# Autodesk Inventor assembly: LR_02
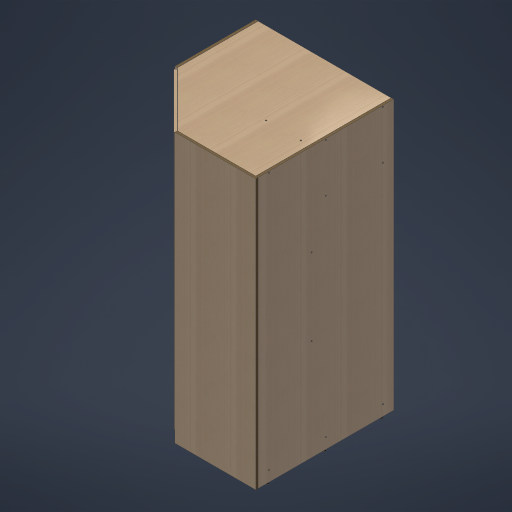
[picture p0: Inventor's stored thumbnail of the model, 512x512]
Saved by Autodesk Inventor 2024.3 (Build 283343000, 343)
## iProperties
Created: 2013-04-02
Part Number: LR_02
Document SubType Name: Assembly
Designer: User
Description: Corner Cabinet
Author: User
## Documents named in this file (23)
- C:\W4INV 2024 Design\PROJECTS\Living Room\Corner Cabinet\LR_02.iam
- C:\W4INV 2024 Design\PROJECTS\Samples\Living Room\Corner Cabinet\LR_0200.ipt
- C:\W4INV 2024 Design\PROJECTS\Samples\Living Room\Corner Cabinet\LR_0203.ipt
- C:\W4INV 2024 Design\PROJECTS\Samples\Living Room\Corner Cabinet\LR_0206.ipt
- C:\W4INV 2024 Design\PROJECTS\Samples\Living Room\Corner Cabinet\LR_0210.ipt
- C:\W4INV 2024 Design\PROJECTS\Samples\Living Room\Corner Cabinet\LR_0201.ipt
- C:\W4INV 2024 Design\PROJECTS\Samples\Living Room\Corner Cabinet\LR_0209.ipt
- C:\W4INV 2024 Design\PROJECTS\Samples\Living Room\Corner Cabinet\LR_0204.ipt
- C:\W4INV 2024 Design\PROJECTS\Samples\Living Room\Corner Cabinet\LR_0205.ipt
- C:\W4INV 2024 Design\PROJECTS\Samples\Living Room\Corner Cabinet\LR_0208.ipt
- C:\W4INV 2024 Design\PROJECTS\Samples\Living Room\Corner Cabinet\LR_0202.ipt
- C:\W4INV 2024 Design\PROJECTS\Samples\Living Room\Corner Cabinet\LR_0207.ipt
- C:\W4INV 2024 Design\_LIBRARY\Fixed joints\Confirmat\CONFIRMAT\Confirmat L50 & Cap D10 NB T18 PB T 18.ipt
- C:\W4INV 2024 Design\_LIBRARY\Fixed joints\Minifix joint\MINIFIX D15 v2\Minifix D15 & Dowel L34 & Cap D15 PB T18 LH.ipt
- C:\W4INV 2024 Design\_LIBRARY\Fixed joints\Minifix joint\MINIFIX D15 v2\Minifix D15 & Dowel L34 & Cap D15 PB T18 RH.ipt
- C:\W4INV 2024 Design\_LIBRARY\Hinges\45 DEGREE HINGE\45 Degree Hinge with Wood Screws And Cup Fixing Wood Screws.iam
- C:\W4INV 2024 Design\_LIBRARY\Supports and legs\Supports\ADJUSTABLE SUPPORT\Support M6 H27 D18 with Bushing SB T18.ipt
- C:\W4INV 2023 Design\LIBRARY\Fixed joints\Confirmat\CONFIRMAT.ipt
- C:\W4INV 2023 Design\LIBRARY\Holders\Shelf holder D5.ipt
- C:\W4INV 2023 Design\LIBRARY\Supports and legs\Supports\ADJUSTABLE SUPPORT.ipt
- C:\W4INV 2023 Design\LIBRARY\Fixed joints\Minifix joint\MINIFIX D15 v2.ipt
- C:\W4INV 2023 Design\LIBRARY\Hinges\45 DEGREE HINGE.iam
- C:\W4INV 2024 Design\_LIBRARY\Holders\Shelf holder D5\Shelf support D5 L16 HOL 3 CAP ON.ipt
## Components (68 placed, 17 different names)
1. LR_0200-Right Side:1 — Flush:1, Flush:2, Mate:135, Mate:141, Mate:180, Mate:188, Mate:192, Mate:200
2. LR_0203-Left Side:1 — Flush:3, Flush:4, Mate:144, Flush:64, Mate:146, Flush:65, Mate:154, Mate:158, Mate:162, Mate:166, Mate:170, Mate:174, Flush:96, Mate:208, Flush:97, Mate:210, Flush:98, Mate:212, Flush:99, Mate:214
3. LR_0206-Back:1 — Mate:91, Flush:38, Mate:93, Flush:39, Mate:95, Flush:40, Mate:97, Flush:41, Mate:99, Flush:42, Mate:101, Flush:43, Flush:48, Flush:49, Mate:115, Flush:50, Mate:117, Flush:51, Mate:147, Mate:148, Flush:66, Mate:149, Mate:150, Flush:67, Mate:151, Mate:152, Flush:68
4. LR_0210-Top:1 — Mate:92, Mate:96, Mate:100, Flush:46, Flush:47, Flush:69, Flush:75, Flush:82, Flush:88
5. LR_0201-Bottom:1 — Mate:94, Mate:98, Mate:102, Flush:73, Flush:79, Flush:86, Flush:92, Flush:93, Flush:95
6. LR_0209-Vertical Partiton:1 — Flush:5, Mate:108, Mate:110, Mate:112, Mate:114, Mate:132, Mate:138, Mate:202, Mate:205
7. LR_0204-Shelve:1 — Mate:116, Mate:118, Flush:71, Flush:77
8. LR_0208-Left Back:1
9. LR_0202-Door:1 — Mate:71, Angle:2, Mate:72, Mate:73, Mate:74
10. LR_0207-Plynth:1
11. Confirmat L50 & Cap D10 NB T18 PB T 18:1 — Mate:91, Mate:92, Flush:38
12. Confirmat L50 & Cap D10 NB T18 PB T 18:2 — Mate:93, Mate:94, Flush:39
13. Confirmat L50 & Cap D10 NB T18 PB T 18:3 — Mate:95, Mate:96, Flush:40
14. Confirmat L50 & Cap D10 NB T18 PB T 18:4 — Mate:97, Mate:98, Flush:41
15. Confirmat L50 & Cap D10 NB T18 PB T 18:5 — Mate:99, Mate:100, Flush:42
16. Confirmat L50 & Cap D10 NB T18 PB T 18:6 — Mate:101, Mate:102, Flush:43
17. Confirmat L50 & Cap D10 NB T18 PB T 18:9 — Mate:107, Flush:46, Mate:108
18. Confirmat L50 & Cap D10 NB T18 PB T 18:10 — Mate:109, Flush:47, Mate:110
19. Confirmat L50 & Cap D10 NB T18 PB T 18:11 — Mate:111, Flush:48, Mate:112
20. Confirmat L50 & Cap D10 NB T18 PB T 18:12 — Mate:113, Flush:49, Mate:114
21. Confirmat L50 & Cap D10 NB T18 PB T 18:13 — Mate:115, Flush:50, Mate:116
22. Confirmat L50 & Cap D10 NB T18 PB T 18:14 — Mate:117, Flush:51, Mate:118
23. Support M6 H27 D18 with Bushing SB T18:6 — Mate:143, Mate:144, Flush:64
24. Support M6 H27 D18 with Bushing SB T18:7 — Mate:145, Mate:146, Flush:65
25. Support M6 H27 D18 with Bushing SB T18:8 — Mate:147, Mate:148, Flush:66
26. Support M6 H27 D18 with Bushing SB T18:9 — Mate:149, Mate:150, Flush:67
27. Support M6 H27 D18 with Bushing SB T18:10 — Mate:151, Mate:152, Flush:68
28. Minifix D15 & Dowel L34 & Cap D15 PB T18 LH:1 — Mate:153, Flush:69, Mate:154
29. Minifix D15 & Dowel L34 & Cap D15 PB T18 RH:3 — Mate:157, Flush:71, Mate:158
30. Minifix D15 & Dowel L34 & Cap D15 PB T18 RH:5 — Mate:161, Flush:73, Mate:162
31. Minifix D15 & Dowel L34 & Cap D15 PB T18 LH:7 — Mate:165, Flush:75, Mate:166
32. Minifix D15 & Dowel L34 & Cap D15 PB T18 LH:9 — Mate:169, Flush:77, Mate:170
33. Minifix D15 & Dowel L34 & Cap D15 PB T18 LH:11 — Mate:173, Flush:79, Mate:174
34. Minifix D15 & Dowel L34 & Cap D15 PB T18 LH:14 — Mate:179, Flush:82, Mate:180
35. Minifix D15 & Dowel L34 & Cap D15 PB T18 RH:18 — Mate:187, Flush:86, Mate:188
36. Minifix D15 & Dowel L34 & Cap D15 PB T18 RH:20 — Mate:191, Flush:88, Mate:192
37. Minifix D15 & Dowel L34 & Cap D15 PB T18 LH:24 — Mate:199, Flush:92, Mate:200
38. Confirmat L50 & Cap D10 NB T18 PB T 18:15 — Mate:201, Flush:93, Mate:202
39. Confirmat L50 & Cap D10 NB T18 PB T 18:17 — Flush:95, Mate:205, Mate:206
40. 45 Degree Hinge with Wood Screws And Cup Fixing Wood Screws:2 [sub-assembly] — Mate:207, Flush:96, Mate:208
41. 45 Degree Hinge with Wood Screws And Cup Fixing Wood Screws:3 [sub-assembly] — Mate:209, Flush:97, Mate:210
42. 45 Degree Hinge with Wood Screws And Cup Fixing Wood Screws:4 [sub-assembly] — Mate:211, Flush:98, Mate:212
43. 45 Degree Hinge with Wood Screws And Cup Fixing Wood Screws:5 [sub-assembly] — Mate:213, Flush:99, Mate:214
44. LR_0205-Shelve:1 — Mate:133, Mate:136, Mate:139, Mate:142
45. Shelf support D5 L16 HOL 3 CAP ON:1 — Mate:131, Mate:132, Mate:133
46. Shelf support D5 L16 HOL 3 CAP ON:3 — Mate:137, Mate:138, Mate:139
47. Shelf support D5 L16 HOL 3 CAP ON:4 — Mate:140, Mate:141, Mate:142
48. Shelf support D5 L16 HOL 3 CAP ON:2 — Mate:134, Mate:135, Mate:136
49. LR_0205-Shelve:2
50. Shelf support D5 L16 HOL 3 CAP ON:5
51. Shelf support D5 L16 HOL 3 CAP ON:6
52. Shelf support D5 L16 HOL 3 CAP ON:7
53. Shelf support D5 L16 HOL 3 CAP ON:8
54. LR_0205-Shelve:3
55. Shelf support D5 L16 HOL 3 CAP ON:9
56. Shelf support D5 L16 HOL 3 CAP ON:10
57. Shelf support D5 L16 HOL 3 CAP ON:11
58. Shelf support D5 L16 HOL 3 CAP ON:12
59. LR_0205-Shelve:4
60. Shelf support D5 L16 HOL 3 CAP ON:13
61. Shelf support D5 L16 HOL 3 CAP ON:14
62. Shelf support D5 L16 HOL 3 CAP ON:15
63. Shelf support D5 L16 HOL 3 CAP ON:16
64. LR_0205-Shelve:5
65. Shelf support D5 L16 HOL 3 CAP ON:17
66. Shelf support D5 L16 HOL 3 CAP ON:18
67. Shelf support D5 L16 HOL 3 CAP ON:19
68. Shelf support D5 L16 HOL 3 CAP ON:20
## Component patterns: (5 elements, first: LR_0205-Shelve:1 + Shelf support D5 L16 HOL 3 CAP ON:1 + Shelf support D5 L16 HOL 3 CAP ON:3 + Shelf support D5 L16 HOL 3 CAP ON:4 + Shelf support D5 L16 HOL 3 CAP ON:2)
## Relationships (124: Mate 82, Flush 38, Angle 4)
- Flush:1 (-80 mm): LR_0200-Right Side:1
- Flush:2 (-80 mm): LR_0200-Right Side:1
- Flush:3 (-80 mm): LR_0203-Left Side:1
- Flush:4 (-80 mm): LR_0203-Left Side:1
- Flush:5 (-80 mm): LR_0209-Vertical Partiton:1
- Mate:71: LR_0202-Door:1
- Angle:2 (0 deg): LR_0202-Door:1
- Mate:72: LR_0202-Door:1
- Angle:3 (0 deg)
- Mate:73: LR_0202-Door:1
- Angle:4 (0 deg)
- Mate:74: LR_0202-Door:1
- Angle:5 (0 deg)
- Mate:91: LR_0206-Back:1 ↔ Confirmat L50 & Cap D10 NB T18 PB T 18:1
- Mate:92 (-9 mm): LR_0210-Top:1 ↔ Confirmat L50 & Cap D10 NB T18 PB T 18:1
- Flush:38: LR_0206-Back:1 ↔ Confirmat L50 & Cap D10 NB T18 PB T 18:1
- Mate:93: LR_0206-Back:1 ↔ Confirmat L50 & Cap D10 NB T18 PB T 18:2
- Mate:94 (-9 mm): LR_0201-Bottom:1 ↔ Confirmat L50 & Cap D10 NB T18 PB T 18:2
- Flush:39: LR_0206-Back:1 ↔ Confirmat L50 & Cap D10 NB T18 PB T 18:2
- Mate:95: LR_0206-Back:1 ↔ Confirmat L50 & Cap D10 NB T18 PB T 18:3
- Mate:96 (-9 mm): LR_0210-Top:1 ↔ Confirmat L50 & Cap D10 NB T18 PB T 18:3
- Flush:40: LR_0206-Back:1 ↔ Confirmat L50 & Cap D10 NB T18 PB T 18:3
- Mate:97: LR_0206-Back:1 ↔ Confirmat L50 & Cap D10 NB T18 PB T 18:4
- Mate:98 (-9 mm): LR_0201-Bottom:1 ↔ Confirmat L50 & Cap D10 NB T18 PB T 18:4
- Flush:41: LR_0206-Back:1 ↔ Confirmat L50 & Cap D10 NB T18 PB T 18:4
- Mate:99: LR_0206-Back:1 ↔ Confirmat L50 & Cap D10 NB T18 PB T 18:5
- Mate:100 (-9 mm): LR_0210-Top:1 ↔ Confirmat L50 & Cap D10 NB T18 PB T 18:5
- Flush:42: LR_0206-Back:1 ↔ Confirmat L50 & Cap D10 NB T18 PB T 18:5
- Mate:101: LR_0206-Back:1 ↔ Confirmat L50 & Cap D10 NB T18 PB T 18:6
- Mate:102 (-9 mm): LR_0201-Bottom:1 ↔ Confirmat L50 & Cap D10 NB T18 PB T 18:6
- Flush:43: LR_0206-Back:1 ↔ Confirmat L50 & Cap D10 NB T18 PB T 18:6
- Mate:107: Confirmat L50 & Cap D10 NB T18 PB T 18:9
- Flush:46: LR_0210-Top:1 ↔ Confirmat L50 & Cap D10 NB T18 PB T 18:9
- Mate:108 (-9 mm): LR_0209-Vertical Partiton:1 ↔ Confirmat L50 & Cap D10 NB T18 PB T 18:9
- Mate:109: Confirmat L50 & Cap D10 NB T18 PB T 18:10
- Flush:47: LR_0210-Top:1 ↔ Confirmat L50 & Cap D10 NB T18 PB T 18:10
- Mate:110 (-9 mm): LR_0209-Vertical Partiton:1 ↔ Confirmat L50 & Cap D10 NB T18 PB T 18:10
- Mate:111: Confirmat L50 & Cap D10 NB T18 PB T 18:11
- Flush:48: LR_0206-Back:1 ↔ Confirmat L50 & Cap D10 NB T18 PB T 18:11
- Mate:112 (-9 mm): LR_0209-Vertical Partiton:1 ↔ Confirmat L50 & Cap D10 NB T18 PB T 18:11
- Mate:113: Confirmat L50 & Cap D10 NB T18 PB T 18:12
- Flush:49: LR_0206-Back:1 ↔ Confirmat L50 & Cap D10 NB T18 PB T 18:12
- Mate:114 (-9 mm): LR_0209-Vertical Partiton:1 ↔ Confirmat L50 & Cap D10 NB T18 PB T 18:12
- Mate:115: LR_0206-Back:1 ↔ Confirmat L50 & Cap D10 NB T18 PB T 18:13
- Flush:50: LR_0206-Back:1 ↔ Confirmat L50 & Cap D10 NB T18 PB T 18:13
- Mate:116 (-9 mm): LR_0204-Shelve:1 ↔ Confirmat L50 & Cap D10 NB T18 PB T 18:13
- Mate:117: LR_0206-Back:1 ↔ Confirmat L50 & Cap D10 NB T18 PB T 18:14
- Flush:51: LR_0206-Back:1 ↔ Confirmat L50 & Cap D10 NB T18 PB T 18:14
- Mate:118 (-9 mm): LR_0204-Shelve:1 ↔ Confirmat L50 & Cap D10 NB T18 PB T 18:14
- Mate:131: Shelf support D5 L16 HOL 3 CAP ON:1
- Mate:132: LR_0209-Vertical Partiton:1 ↔ Shelf support D5 L16 HOL 3 CAP ON:1
- Mate:133 (2.5 mm): LR_0205-Shelve:1 ↔ Shelf support D5 L16 HOL 3 CAP ON:1
- Mate:134: Shelf support D5 L16 HOL 3 CAP ON:2
- Mate:135: LR_0200-Right Side:1 ↔ Shelf support D5 L16 HOL 3 CAP ON:2
- Mate:136 (2.5 mm): LR_0205-Shelve:1 ↔ Shelf support D5 L16 HOL 3 CAP ON:2
- Mate:137: Shelf support D5 L16 HOL 3 CAP ON:3
- Mate:138: LR_0209-Vertical Partiton:1 ↔ Shelf support D5 L16 HOL 3 CAP ON:3
- Mate:139 (2.5 mm): LR_0205-Shelve:1 ↔ Shelf support D5 L16 HOL 3 CAP ON:3
- Mate:140: Shelf support D5 L16 HOL 3 CAP ON:4
- Mate:141: LR_0200-Right Side:1 ↔ Shelf support D5 L16 HOL 3 CAP ON:4
- Mate:142 (2.5 mm): LR_0205-Shelve:1 ↔ Shelf support D5 L16 HOL 3 CAP ON:4
- Mate:143: Support M6 H27 D18 with Bushing SB T18:6
- Mate:144 (17.5 mm): LR_0203-Left Side:1 ↔ Support M6 H27 D18 with Bushing SB T18:6
- Flush:64 (9 mm): LR_0203-Left Side:1 ↔ Support M6 H27 D18 with Bushing SB T18:6
- Mate:145: Support M6 H27 D18 with Bushing SB T18:7
- Mate:146 (17.5 mm): LR_0203-Left Side:1 ↔ Support M6 H27 D18 with Bushing SB T18:7
- Flush:65 (9 mm): LR_0203-Left Side:1 ↔ Support M6 H27 D18 with Bushing SB T18:7
- Mate:147: LR_0206-Back:1 ↔ Support M6 H27 D18 with Bushing SB T18:8
- Mate:148 (17.5 mm): LR_0206-Back:1 ↔ Support M6 H27 D18 with Bushing SB T18:8
- Flush:66 (9 mm): LR_0206-Back:1 ↔ Support M6 H27 D18 with Bushing SB T18:8
- Mate:149: LR_0206-Back:1 ↔ Support M6 H27 D18 with Bushing SB T18:9
- Mate:150 (17.5 mm): LR_0206-Back:1 ↔ Support M6 H27 D18 with Bushing SB T18:9
- Flush:67 (9 mm): LR_0206-Back:1 ↔ Support M6 H27 D18 with Bushing SB T18:9
- Mate:151: LR_0206-Back:1 ↔ Support M6 H27 D18 with Bushing SB T18:10
- Mate:152 (17.5 mm): LR_0206-Back:1 ↔ Support M6 H27 D18 with Bushing SB T18:10
- Flush:68 (9 mm): LR_0206-Back:1 ↔ Support M6 H27 D18 with Bushing SB T18:10
- Mate:153: Minifix D15 & Dowel L34 & Cap D15 PB T18 LH:1
- Flush:69 (18 mm): LR_0210-Top:1 ↔ Minifix D15 & Dowel L34 & Cap D15 PB T18 LH:1
- Mate:154: LR_0203-Left Side:1 ↔ Minifix D15 & Dowel L34 & Cap D15 PB T18 LH:1
- Mate:157: Minifix D15 & Dowel L34 & Cap D15 PB T18 RH:3
- Flush:71 (18 mm): LR_0204-Shelve:1 ↔ Minifix D15 & Dowel L34 & Cap D15 PB T18 RH:3
- Mate:158: LR_0203-Left Side:1 ↔ Minifix D15 & Dowel L34 & Cap D15 PB T18 RH:3
- Mate:161: Minifix D15 & Dowel L34 & Cap D15 PB T18 RH:5
- Flush:73 (18 mm): LR_0201-Bottom:1 ↔ Minifix D15 & Dowel L34 & Cap D15 PB T18 RH:5
- Mate:162: LR_0203-Left Side:1 ↔ Minifix D15 & Dowel L34 & Cap D15 PB T18 RH:5
- Mate:165: Minifix D15 & Dowel L34 & Cap D15 PB T18 LH:7
- Flush:75 (18 mm): LR_0210-Top:1 ↔ Minifix D15 & Dowel L34 & Cap D15 PB T18 LH:7
- Mate:166: LR_0203-Left Side:1 ↔ Minifix D15 & Dowel L34 & Cap D15 PB T18 LH:7
- Mate:169: Minifix D15 & Dowel L34 & Cap D15 PB T18 LH:9
- Flush:77 (18 mm): LR_0204-Shelve:1 ↔ Minifix D15 & Dowel L34 & Cap D15 PB T18 LH:9
- Mate:170: LR_0203-Left Side:1 ↔ Minifix D15 & Dowel L34 & Cap D15 PB T18 LH:9
- Mate:173: Minifix D15 & Dowel L34 & Cap D15 PB T18 LH:11
- Flush:79 (18 mm): LR_0201-Bottom:1 ↔ Minifix D15 & Dowel L34 & Cap D15 PB T18 LH:11
- Mate:174: LR_0203-Left Side:1 ↔ Minifix D15 & Dowel L34 & Cap D15 PB T18 LH:11
- Mate:179: Minifix D15 & Dowel L34 & Cap D15 PB T18 LH:14
- Flush:82 (18 mm): LR_0210-Top:1 ↔ Minifix D15 & Dowel L34 & Cap D15 PB T18 LH:14
- Mate:180: LR_0200-Right Side:1 ↔ Minifix D15 & Dowel L34 & Cap D15 PB T18 LH:14
- Mate:187: Minifix D15 & Dowel L34 & Cap D15 PB T18 RH:18
- Flush:86 (18 mm): LR_0201-Bottom:1 ↔ Minifix D15 & Dowel L34 & Cap D15 PB T18 RH:18
- Mate:188: LR_0200-Right Side:1 ↔ Minifix D15 & Dowel L34 & Cap D15 PB T18 RH:18
- Mate:191: Minifix D15 & Dowel L34 & Cap D15 PB T18 RH:20
- Flush:88 (18 mm): LR_0210-Top:1 ↔ Minifix D15 & Dowel L34 & Cap D15 PB T18 RH:20
- Mate:192: LR_0200-Right Side:1 ↔ Minifix D15 & Dowel L34 & Cap D15 PB T18 RH:20
- Mate:199: Minifix D15 & Dowel L34 & Cap D15 PB T18 LH:24
- Flush:92 (18 mm): LR_0201-Bottom:1 ↔ Minifix D15 & Dowel L34 & Cap D15 PB T18 LH:24
- Mate:200: LR_0200-Right Side:1 ↔ Minifix D15 & Dowel L34 & Cap D15 PB T18 LH:24
- Mate:201: Confirmat L50 & Cap D10 NB T18 PB T 18:15
- Flush:93: LR_0201-Bottom:1 ↔ Confirmat L50 & Cap D10 NB T18 PB T 18:15
- Mate:202 (-9 mm): LR_0209-Vertical Partiton:1 ↔ Confirmat L50 & Cap D10 NB T18 PB T 18:15
- Flush:95: LR_0201-Bottom:1 ↔ Confirmat L50 & Cap D10 NB T18 PB T 18:17
- Mate:205 (-9 mm): LR_0209-Vertical Partiton:1 ↔ Confirmat L50 & Cap D10 NB T18 PB T 18:17
- Mate:206: Confirmat L50 & Cap D10 NB T18 PB T 18:17
- Mate:207: 45 Degree Hinge with Wood Screws And Cup Fixing Wood Screws:2
- Flush:96 (37 mm): LR_0203-Left Side:1 ↔ 45 Degree Hinge with Wood Screws And Cup Fixing Wood Screws:2
- Mate:208: LR_0203-Left Side:1 ↔ 45 Degree Hinge with Wood Screws And Cup Fixing Wood Screws:2
- Mate:209: 45 Degree Hinge with Wood Screws And Cup Fixing Wood Screws:3
- Flush:97 (37 mm): LR_0203-Left Side:1 ↔ 45 Degree Hinge with Wood Screws And Cup Fixing Wood Screws:3
- Mate:210: LR_0203-Left Side:1 ↔ 45 Degree Hinge with Wood Screws And Cup Fixing Wood Screws:3
- Mate:211: 45 Degree Hinge with Wood Screws And Cup Fixing Wood Screws:4
- Flush:98 (37 mm): LR_0203-Left Side:1 ↔ 45 Degree Hinge with Wood Screws And Cup Fixing Wood Screws:4
- Mate:212: LR_0203-Left Side:1 ↔ 45 Degree Hinge with Wood Screws And Cup Fixing Wood Screws:4
- Mate:213: 45 Degree Hinge with Wood Screws And Cup Fixing Wood Screws:5
- Flush:99 (37 mm): LR_0203-Left Side:1 ↔ 45 Degree Hinge with Wood Screws And Cup Fixing Wood Screws:5
- Mate:214: LR_0203-Left Side:1 ↔ 45 Degree Hinge with Wood Screws And Cup Fixing Wood Screws:5
